# Autodesk Inventor assembly: Water system
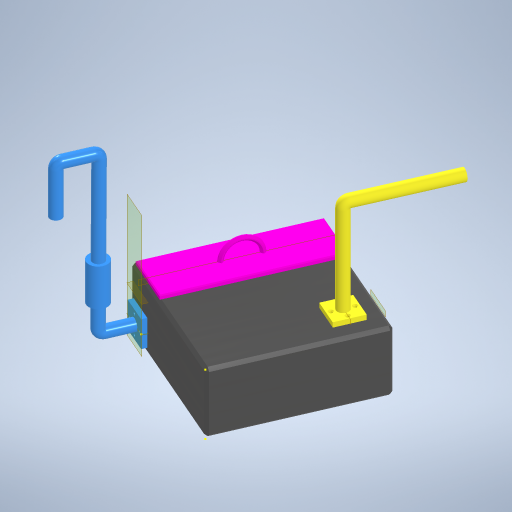
[picture p0: Inventor's stored thumbnail of the model, 512x512]
Saved by Autodesk Inventor 2023 (Build 270158000, 158)
## iProperties
Created: 2022-11-25
Part Number: Water system
Document SubType Name: Assembly
Designer: hp
Author: hp
## Documents named in this file (5)
- C:\Users\hp\Downloads\Water system.iam
- C:\Users\hp\Desktop\Coffee\Coffee course\Water container.ipt
- C:\Users\hp\Desktop\Coffee\Coffee course\water lock.ipt
- C:\Users\hp\Desktop\Coffee\Coffee course\water tube to pump.ipt
- C:\Users\hp\Desktop\Coffee\Coffee course\water to water container.ipt
## Components (4 placed, 4 different names)
1. Water container:1 — Mate:1, Mate:2, Mate:3, Mate:4, Mate:5, Mate:6, Mate:7, Mate:8
2. water lock:1 — Mate:1, Mate:2, Mate:3
3. water tube to pump:1 — Mate:4, Mate:5
4. water to water container:1 — Mate:6, Mate:7, Mate:8
## Relationships (8: Mate 8)
- Mate:1: Water container:1 ↔ water lock:1
- Mate:2: Water container:1 ↔ water lock:1
- Mate:3: Water container:1 ↔ water lock:1
- Mate:4: Water container:1 ↔ water tube to pump:1
- Mate:5: Water container:1 ↔ water tube to pump:1
- Mate:6: Water container:1 ↔ water to water container:1
- Mate:7: Water container:1 ↔ water to water container:1
- Mate:8: Water container:1 ↔ water to water container:1
